# Autodesk Inventor assembly: CAM2
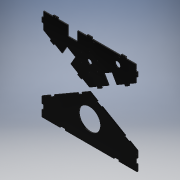
[picture p0: Inventor's stored thumbnail of the model, 180x180]
Saved by Autodesk Inventor 2017 (Build 210142000, 142)
## iProperties
Created: 2019-05-25
Part Number: CAM2
Document SubType Name: Assembly
Designer: 3D Printer
Author: 3D Printer
## Documents named in this file (3)
- C:\Users\Dell\Documents\GitHub\tr2\Body 2.0\CAM2.iam
- C:\Users\Dell\Documents\GitHub\tr2\Body 2.0\BA01.ipt
- C:\Users\Dell\Documents\GitHub\tr2\Body 2.0\BA08.ipt
## Components (2 placed, 2 different names)
1. BA01:1 — Mate:1, Mate:4, Mate:5, Angle:1, Mate:6, Flush:1
2. BA08:1 — Mate:3, Mate:5, Angle:1, Flush:1
## Relationships (7: Mate 5, Angle 1, Flush 1)
- Mate:1: BA01:1
- Mate:3: BA08:1
- Mate:4: BA01:1
- Mate:5 (20 mm): BA01:1 ↔ BA08:1
- Angle:1 (0 deg): BA01:1 ↔ BA08:1
- Mate:6: BA01:1
- Flush:1: BA01:1 ↔ BA08:1
